# Autodesk Inventor assembly: Non-Rotating Carousel Assembly
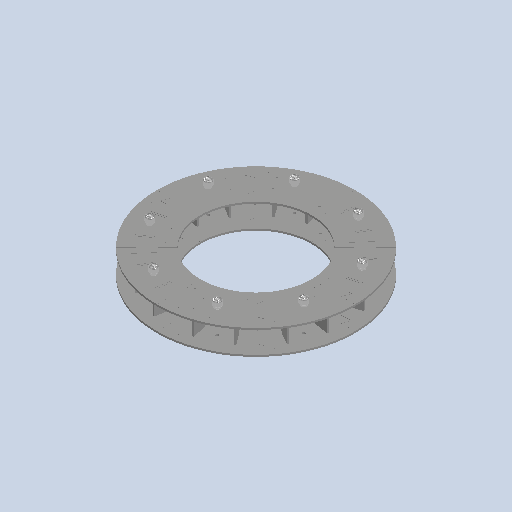
[picture p0: Inventor's stored thumbnail of the model, 512x512]
Saved by Autodesk Inventor 2023 (Build 270158000, 158)
## iProperties
Created: 2023-02-13
Part Number: Non-Rotating Carousel Assembly
Document SubType Name: Assembly
Designer: cheng
Mass: 2761.42 g
Surface Area: 9446.3 cm^2
Volume: 2045.26 cm^3
Density: 1.35016 g/cm^3
Author: cheng
## Documents named in this file (2)
- C:\Users\mihal\Desktop\4th Year Project\Final Assembly\Carousel Base Plate Laser Cut\Non-Rotating Carousel Assembly.iam
- C:\Users\mihal\Desktop\4th Year Project\Final Assembly\Carousel Base Plate Laser Cut\Non-Rotating Carousel Section Assembly.iam
## Components (8 placed, 1 different names)
1. Non-Rotating Carousel Section Assembly:1 [sub-assembly] — Mate:7, Flush:4, Mate:8
2. Non-Rotating Carousel Section Assembly:2 [sub-assembly] — Mate:13, Mate:14, Flush:7
3. Non-Rotating Carousel Section Assembly:3 [sub-assembly] — Mate:9, Mate:10, Flush:5, Mate:11, Mate:12, Flush:6, Mate:16
4. Non-Rotating Carousel Section Assembly:4 [sub-assembly] — Mate:11, Mate:12, Flush:6, Mate:13, Mate:14, Flush:7
5. Non-Rotating Carousel Section Assembly:5 [sub-assembly] — Flush:2, Mate:3, Mate:4, Mate:5, Flush:3, Mate:6
6. Non-Rotating Carousel Section Assembly:6 [sub-assembly] — Mate:5, Flush:3, Mate:6, Mate:7, Flush:4, Mate:8
7. Non-Rotating Carousel Section Assembly:7 [sub-assembly] — Mate:1, Mate:2, Flush:1, Mate:9, Mate:10, Flush:5, Mate:15
8. Non-Rotating Carousel Section Assembly:8 [sub-assembly] — Mate:1, Mate:2, Flush:1, Flush:2, Mate:3, Mate:4
## Relationships (23: Mate 16, Flush 7)
- Mate:1: Non-Rotating Carousel Section Assembly:7 ↔ Non-Rotating Carousel Section Assembly:8
- Mate:2: Non-Rotating Carousel Section Assembly:7 ↔ Non-Rotating Carousel Section Assembly:8
- Flush:1: Non-Rotating Carousel Section Assembly:7 ↔ Non-Rotating Carousel Section Assembly:8
- Flush:2: Non-Rotating Carousel Section Assembly:5 ↔ Non-Rotating Carousel Section Assembly:8
- Mate:3: Non-Rotating Carousel Section Assembly:5 ↔ Non-Rotating Carousel Section Assembly:8
- Mate:4: Non-Rotating Carousel Section Assembly:5 ↔ Non-Rotating Carousel Section Assembly:8
- Mate:5: Non-Rotating Carousel Section Assembly:5 ↔ Non-Rotating Carousel Section Assembly:6
- Flush:3: Non-Rotating Carousel Section Assembly:5 ↔ Non-Rotating Carousel Section Assembly:6
- Mate:6: Non-Rotating Carousel Section Assembly:5 ↔ Non-Rotating Carousel Section Assembly:6
- Mate:7: Non-Rotating Carousel Section Assembly:1 ↔ Non-Rotating Carousel Section Assembly:6
- Flush:4: Non-Rotating Carousel Section Assembly:1 ↔ Non-Rotating Carousel Section Assembly:6
- Mate:8: Non-Rotating Carousel Section Assembly:1 ↔ Non-Rotating Carousel Section Assembly:6
- Mate:9: Non-Rotating Carousel Section Assembly:3 ↔ Non-Rotating Carousel Section Assembly:7
- Mate:10: Non-Rotating Carousel Section Assembly:3 ↔ Non-Rotating Carousel Section Assembly:7
- Flush:5: Non-Rotating Carousel Section Assembly:3 ↔ Non-Rotating Carousel Section Assembly:7
- Mate:11: Non-Rotating Carousel Section Assembly:3 ↔ Non-Rotating Carousel Section Assembly:4
- Mate:12: Non-Rotating Carousel Section Assembly:3 ↔ Non-Rotating Carousel Section Assembly:4
- Flush:6: Non-Rotating Carousel Section Assembly:3 ↔ Non-Rotating Carousel Section Assembly:4
- Mate:13: Non-Rotating Carousel Section Assembly:2 ↔ Non-Rotating Carousel Section Assembly:4
- Mate:14: Non-Rotating Carousel Section Assembly:2 ↔ Non-Rotating Carousel Section Assembly:4
- Flush:7: Non-Rotating Carousel Section Assembly:2 ↔ Non-Rotating Carousel Section Assembly:4
- Mate:15: Non-Rotating Carousel Section Assembly:7
- Mate:16: Non-Rotating Carousel Section Assembly:3
